# Autodesk Inventor assembly: HalfTop
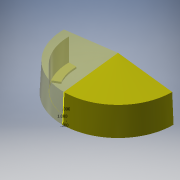
[picture p0: Inventor's stored thumbnail of the model, 180x180]
Saved by Autodesk Inventor 2019 (Build 230136000, 136)
## iProperties
Created: 2019-10-06
Part Number: HalfTop
Document SubType Name: Assembly
Designer: james
Author: james
## Documents named in this file (3)
- F:\JimsDesign\Jims2020FTC\HalfTop.iam
- F:\JimsDesign\Jims2020FTC\QuarterTop2.ipt
- F:\JimsDesign\Jims2020FTC\QuarterTop.ipt
## Components (2 placed, 2 different names)
1. QuarterTop2:1 — Mate:1, Flush:1, Flush:2
2. QuarterTop:1 — Mate:1, Flush:1, Flush:2
## Relationships (3: Flush 2, Mate 1)
- Mate:1: QuarterTop2:1 ↔ QuarterTop:1
- Flush:1: QuarterTop2:1 ↔ QuarterTop:1
- Flush:2: QuarterTop2:1 ↔ QuarterTop:1
